# Autodesk Inventor assembly: Hip Long
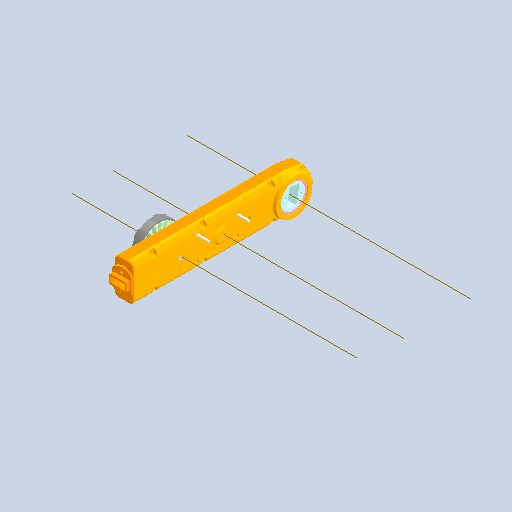
[picture p0: Inventor's stored thumbnail of the model, 512x512]
Saved by Autodesk Inventor 2022.2 (Build 262287030, 287C)
## iProperties
Created: 2022-01-09
Part Number: Hip Long
Document SubType Name: Assembly
Designer: Jochen
Author: Jochen
## Documents named in this file (10)
- D:\Projects\Lisbeth\CAD\Hip\Hip Long.iam
- D:\Projects\Lisbeth\CAD\Common\Motor\MotorModule.iam
- D:\Projects\Lisbeth\CAD\Common\Encoder\encoder.iam
- D:\Projects\Lisbeth\CAD\Common\Transmission\TransmissionPulleyCenter.iam
- D:\Projects\Lisbeth\CAD\Common\Transmission\Transmission Pulley.iam
- D:\Projects\Lisbeth\CAD\Common\Belt Tensioner\BeltTensioner 10mm.iam
- D:\Projects\Lisbeth\CAD\Common\Belt Tensioner\MotorBeltTensioner 10mm.iam
- D:\Projects\Lisbeth\CAD\Hip\Hip\Design Accelerator\Synchronous Belts Transmission1.iam
- D:\Projects\Lisbeth\CAD\Hip\Hip\Design Accelerator\Synchronous Belts Transmission2.iam
- D:\Projects\Lisbeth\CAD\Hip\HipBody Long.ipt
## Components (9 placed, 8 different names)
1. MotorModule:2 [sub-assembly] — Mate:3, Mate:4
2. Encoder:2 [sub-assembly] — Angle:1
3. TransmissionPuileyCenter:1 [sub-assembly] — Mate:5, Mate:6
4. Transmission Pulley:1 [sub-assembly] — Mate:1, Mate:2
5. Belt tensioner:1 [sub-assembly]
6. MotorBeltTensioner:1 [sub-assembly]
7. Synchronous Belts Transmission:1 [sub-assembly]
8. Synchronous Belts Transmission:2 [sub-assembly]
9. HipBody:1 — Mate:1, Mate:2, Mate:3, Mate:4, Mate:5, Mate:6
## Relationships (7: Mate 6, Angle 1)
- Angle:1 (0 deg): Encoder:2
- Mate:1: Transmission Pulley:1 ↔ HipBody:1
- Mate:2: Transmission Pulley:1 ↔ HipBody:1
- Mate:3: MotorModule:2 ↔ HipBody:1
- Mate:4: MotorModule:2 ↔ HipBody:1
- Mate:5: TransmissionPuileyCenter:1 ↔ HipBody:1
- Mate:6: TransmissionPuileyCenter:1 ↔ HipBody:1
